# Autodesk Inventor assembly: Clamp with Piston Assembly
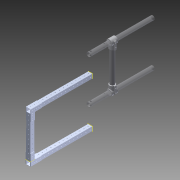
[picture p0: Inventor's stored thumbnail of the model, 180x180]
Saved by Autodesk Inventor 2014 (Build 180170000, 170)
## iProperties
Created: 2014-01-12
Part Number: Clamp with Piston Assembly
Document SubType Name: Assembly
Designer: Michael
Mass: 304.85 g
Surface Area: 1790.43 cm^2
Volume: 181.397 cm^3
Density: 1.68057 g/cm^3
Author: Michael
## Documents named in this file (7)
- C:\Users\Michael\Documents\GitHub\2014buildCAD\New Collector\Clamp with Piston Assembly.iam
- C:\Users\Michael\Documents\GitHub\2014buildCAD\Collector\Polycarbonate Clamp Tube (Middle) (8585K14).ipt
- C:\Users\Michael\Documents\GitHub\2014buildCAD\Collector\Polycarbonate Clamp Tube 1 in OD (8585K14).ipt
- C:\Users\Michael\Documents\GitHub\2014buildCAD\Collector\Metal Pipe T Joint (4698T140).ipt
- C:\Users\Michael\Documents\GitHub\2014buildCAD\New Collector\Vex Pro 1x1 rectangular tubing 10 in length.ipt
- C:\Users\Michael\Documents\GitHub\2014buildCAD\New Collector\Vex Pro 1x1 rectangular tubing 14 in length.ipt
- C:\Users\Michael\Documents\GitHub\2014buildCAD\New Collector\Vex Pro 90 degree gusset.ipt
## Components (12 placed, 6 different names)
1. Polycarbonate Clamp Tube (Middle) (8585K14):1 — Mate:13, Mate:18, Mate:19
2. Polycarbonate Clamp Tube 1 in OD (8585K14):1 — Flush:1, Mate:20, Mate:22
3. Polycarbonate Clamp Tube 1 in OD (8585K14):2 — Mate:21, Mate:22
4. Metal Pipe T Joint (4698T140):1 — Mate:13, Mate:17, Mate:18, Mate:21
5. Metal Pipe T Joint (4698T140):2 — Mate:17, Mate:19, Flush:1, Mate:20
6. Vex Pro 1x1 rectangular tubing 10 in length:1 — Mate:29, Mate:30, Mate:31, Mate:32, Mate:33, Mate:34, Mate:35, Mate:36, Mate:46
7. Vex Pro 1x1 rectangular tubing 14 in length:1 — Mate:23, Mate:26, Mate:40, Mate:41, Mate:42, Mate:43
8. Vex Pro 1x1 rectangular tubing 14 in length:2 — Mate:39, Mate:44, Mate:45
9. Vex Pro 90 degree gusset:1 — Mate:35, Mate:36, Mate:39, Mate:46
10. Vex Pro 90 degree gusset:2 — Mate:23, Mate:29, Mate:30, Mate:40, Mate:41
11. Vex Pro 90 degree gusset:3 — Mate:26, Mate:31, Mate:42, Mate:43
12. Vex Pro 90 degree gusset:4 — Mate:32, Mate:33, Mate:34, Mate:44, Mate:45
## Relationships (26: Mate 25, Flush 1)
- Mate:13: Polycarbonate Clamp Tube (Middle) (8585K14):1 ↔ Metal Pipe T Joint (4698T140):1
- Mate:17 (188.976 mm): Metal Pipe T Joint (4698T140):1 ↔ Metal Pipe T Joint (4698T140):2
- Mate:18 (-12.7 mm): Polycarbonate Clamp Tube (Middle) (8585K14):1 ↔ Metal Pipe T Joint (4698T140):1
- Mate:19: Polycarbonate Clamp Tube (Middle) (8585K14):1 ↔ Metal Pipe T Joint (4698T140):2
- Flush:1 (127 mm): Polycarbonate Clamp Tube 1 in OD (8585K14):1 ↔ Metal Pipe T Joint (4698T140):2
- Mate:20: Polycarbonate Clamp Tube 1 in OD (8585K14):1 ↔ Metal Pipe T Joint (4698T140):2
- Mate:21: Polycarbonate Clamp Tube 1 in OD (8585K14):2 ↔ Metal Pipe T Joint (4698T140):1
- Mate:22: Polycarbonate Clamp Tube 1 in OD (8585K14):1 ↔ Polycarbonate Clamp Tube 1 in OD (8585K14):2
- Mate:23: Vex Pro 1x1 rectangular tubing 14 in length:1 ↔ Vex Pro 90 degree gusset:2
- Mate:26: Vex Pro 1x1 rectangular tubing 14 in length:1 ↔ Vex Pro 90 degree gusset:3
- Mate:29: Vex Pro 1x1 rectangular tubing 10 in length:1 ↔ Vex Pro 90 degree gusset:2
- Mate:30: Vex Pro 1x1 rectangular tubing 10 in length:1 ↔ Vex Pro 90 degree gusset:2
- Mate:31: Vex Pro 1x1 rectangular tubing 10 in length:1 ↔ Vex Pro 90 degree gusset:3
- Mate:32: Vex Pro 1x1 rectangular tubing 10 in length:1 ↔ Vex Pro 90 degree gusset:4
- Mate:33: Vex Pro 1x1 rectangular tubing 10 in length:1 ↔ Vex Pro 90 degree gusset:4
- Mate:34: Vex Pro 1x1 rectangular tubing 10 in length:1 ↔ Vex Pro 90 degree gusset:4
- Mate:35: Vex Pro 1x1 rectangular tubing 10 in length:1 ↔ Vex Pro 90 degree gusset:1
- Mate:36: Vex Pro 1x1 rectangular tubing 10 in length:1 ↔ Vex Pro 90 degree gusset:1
- Mate:39: Vex Pro 1x1 rectangular tubing 14 in length:2 ↔ Vex Pro 90 degree gusset:1
- Mate:40: Vex Pro 1x1 rectangular tubing 14 in length:1 ↔ Vex Pro 90 degree gusset:2
- Mate:41: Vex Pro 1x1 rectangular tubing 14 in length:1 ↔ Vex Pro 90 degree gusset:2
- Mate:42: Vex Pro 1x1 rectangular tubing 14 in length:1 ↔ Vex Pro 90 degree gusset:3
- Mate:43: Vex Pro 1x1 rectangular tubing 14 in length:1 ↔ Vex Pro 90 degree gusset:3
- Mate:44: Vex Pro 1x1 rectangular tubing 14 in length:2 ↔ Vex Pro 90 degree gusset:4
- Mate:45: Vex Pro 1x1 rectangular tubing 14 in length:2 ↔ Vex Pro 90 degree gusset:4
- Mate:46: Vex Pro 1x1 rectangular tubing 10 in length:1 ↔ Vex Pro 90 degree gusset:1
